# Autodesk Inventor assembly: scissor
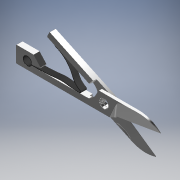
[picture p0: Inventor's stored thumbnail of the model, 180x180]
Saved by Autodesk Inventor 2019 (Build 230136000, 136)
## iProperties
Shininess: 0.0
Length Units: 11269
Angle Units: 11279
Time Units: 11290
Mass Units: 11283
Length Display Precision: 3
Angle Display Precision: 2
Compacted: True
Company: Autodesk
Created: 2000-05-30
Part Number: scissor
Document SubType Name: Assembly
Designer: Autodesk, Inc.
Mass: 2.59142 g
Surface Area: 10.2944 cm^2
Volume: 0.334133 cm^3
Density: 7.75563 g/cm^3
Density: 0.0
Volumn: 0.0
Area: 0.0
PropertySet Name: Model Information
Control State: 0
Master: False
Checked Out: False
Subject: Inventor Samples
Author: Autodesk, Inc.
## Documents named in this file (4)
- C:\Users\itools\Desktop\autodesk_inventor_2018_samples\Models\Assemblies\Scissors\scissors.iam
- C:\Users\itools\Desktop\autodesk_inventor_2018_samples\Models\Assemblies\Scissors\Components\blade_main.ipt
- C:\Users\itools\Desktop\autodesk_inventor_2018_samples\Models\Assemblies\Scissors\Components\blade_top.ipt
- C:\Users\itools\Desktop\autodesk_inventor_2018_samples\Models\Assemblies\Scissors\Components\scissor_spring.ipt
## Components (3 placed, 3 different names)
1. blade_main:1 — Insert:1, Insert:2, Mate:1, Angle:1
2. blade_top:1 — Insert:1, Tangent:1, Angle:1
3. scissor_spring:1 — Insert:2, Mate:1, Tangent:1
## Relationships (5: Insert 2, Mate 1, Tangent 1, Angle 1)
- Insert:1: blade_main:1 ↔ blade_top:1
- Insert:2: blade_main:1 ↔ scissor_spring:1
- Mate:1: blade_main:1 ↔ scissor_spring:1
- Tangent:1: blade_top:1 ↔ scissor_spring:1
- Angle:1 (155 deg): blade_main:1 ↔ blade_top:1
